(part 1 of 2)
# Autodesk Inventor assembly: Raspberry Pi 3
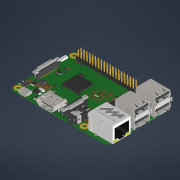
[picture p0: Inventor's stored thumbnail of the model, 180x180]
Saved by Autodesk Inventor 2021 (Build 250183000, 183)
## iProperties
Created: 2016-07-31
Part Number: Raspberry Pi 3
Document SubType Name: Assembly
Designer: sbahn
Author: sbahn
Sending System: SolidWorks 2016
Last Author: awillame
Last Saved: 2017-12-17
## Documents named in this file (329)
- C:\Users\sbahn\Desktop\개인자료\Workspace\Python Workspace\고등학교 졸업과제\2학기\modeling\electronic_file\raspi\Raspberry Pi 3.iam
- C:\Users\sbahn\Desktop\개인자료\Workspace\Python Workspace\고등학교 졸업과제\2학기\modeling\electronic_file\raspi\Raspberry Pi 3157.ipt
- C:\Users\sbahn\Desktop\개인자료\Workspace\Python Workspace\고등학교 졸업과제\2학기\modeling\electronic_file\raspi\Raspberry Pi 3242.ipt
- C:\Users\sbahn\Desktop\개인자료\Workspace\Python Workspace\고등학교 졸업과제\2학기\modeling\electronic_file\raspi\Raspberry Pi 3266.ipt
- C:\Users\sbahn\Desktop\개인자료\Workspace\Python Workspace\고등학교 졸업과제\2학기\modeling\electronic_file\raspi\raspberry_pi_3(bar_180_2x20).ipt
- C:\Users\sbahn\Desktop\개인자료\Workspace\Python Workspace\고등학교 졸업과제\2학기\modeling\electronic_file\raspi\RPi3_ModelB v1.iam
- C:\Users\sbahn\Desktop\개인자료\Workspace\Python Workspace\고등학교 졸업과제\2학기\modeling\electronic_file\raspi\Raspberry Pi 312.ipt
- C:\Users\sbahn\Desktop\개인자료\Workspace\Python Workspace\고등학교 졸업과제\2학기\modeling\electronic_file\raspi\Raspberry Pi 314.ipt
- C:\Users\sbahn\Desktop\개인자료\Workspace\Python Workspace\고등학교 졸업과제\2학기\modeling\electronic_file\raspi\Raspberry Pi 3172.ipt
- C:\Users\sbahn\Desktop\개인자료\Workspace\Python Workspace\고등학교 졸업과제\2학기\modeling\electronic_file\raspi\Raspberry Pi 3173.ipt
- C:\Users\sbahn\Desktop\개인자료\Workspace\Python Workspace\고등학교 졸업과제\2학기\modeling\electronic_file\raspi\Raspberry Pi 3174.ipt
- C:\Users\sbahn\Desktop\개인자료\Workspace\Python Workspace\고등학교 졸업과제\2학기\modeling\electronic_file\raspi\Raspberry Pi 3175.ipt
- C:\Users\sbahn\Desktop\개인자료\Workspace\Python Workspace\고등학교 졸업과제\2학기\modeling\electronic_file\raspi\Raspberry Pi 3176.ipt
- C:\Users\sbahn\Desktop\개인자료\Workspace\Python Workspace\고등학교 졸업과제\2학기\modeling\electronic_file\raspi\Raspberry Pi 3177.ipt
- C:\Users\sbahn\Desktop\개인자료\Workspace\Python Workspace\고등학교 졸업과제\2학기\modeling\electronic_file\raspi\Raspberry Pi 3178.ipt
- C:\Users\sbahn\Desktop\개인자료\Workspace\Python Workspace\고등학교 졸업과제\2학기\modeling\electronic_file\raspi\Raspberry Pi 3179.ipt
- C:\Users\sbahn\Desktop\개인자료\Workspace\Python Workspace\고등학교 졸업과제\2학기\modeling\electronic_file\raspi\Raspberry Pi 3180.ipt
- C:\Users\sbahn\Desktop\개인자료\Workspace\Python Workspace\고등학교 졸업과제\2학기\modeling\electronic_file\raspi\Raspberry Pi 3181.ipt
- C:\Users\sbahn\Desktop\개인자료\Workspace\Python Workspace\고등학교 졸업과제\2학기\modeling\electronic_file\raspi\Raspberry Pi 3182.ipt
- C:\Users\sbahn\Desktop\개인자료\Workspace\Python Workspace\고등학교 졸업과제\2학기\modeling\electronic_file\raspi\Raspberry Pi 3183.ipt
- C:\Users\sbahn\Desktop\개인자료\Workspace\Python Workspace\고등학교 졸업과제\2학기\modeling\electronic_file\raspi\Raspberry Pi 3184.ipt
- C:\Users\sbahn\Desktop\개인자료\Workspace\Python Workspace\고등학교 졸업과제\2학기\modeling\electronic_file\raspi\Raspberry Pi 3185.ipt
- C:\Users\sbahn\Desktop\개인자료\Workspace\Python Workspace\고등학교 졸업과제\2학기\modeling\electronic_file\raspi\Raspberry Pi 3186.ipt
- C:\Users\sbahn\Desktop\개인자료\Workspace\Python Workspace\고등학교 졸업과제\2학기\modeling\electronic_file\raspi\Raspberry Pi 3187.ipt
- C:\Users\sbahn\Desktop\개인자료\Workspace\Python Workspace\고등학교 졸업과제\2학기\modeling\electronic_file\raspi\Raspberry Pi 3188.ipt
- C:\Users\sbahn\Desktop\개인자료\Workspace\Python Workspace\고등학교 졸업과제\2학기\modeling\electronic_file\raspi\Raspberry Pi 3189.ipt
- C:\Users\sbahn\Desktop\개인자료\Workspace\Python Workspace\고등학교 졸업과제\2학기\modeling\electronic_file\raspi\Raspberry Pi 3190.ipt
- C:\Users\sbahn\Desktop\개인자료\Workspace\Python Workspace\고등학교 졸업과제\2학기\modeling\electronic_file\raspi\Raspberry Pi 3191.ipt
- C:\Users\sbahn\Desktop\개인자료\Workspace\Python Workspace\고등학교 졸업과제\2학기\modeling\electronic_file\raspi\Raspberry Pi 3192.ipt
- C:\Users\sbahn\Desktop\개인자료\Workspace\Python Workspace\고등학교 졸업과제\2학기\modeling\electronic_file\raspi\Raspberry Pi 3193.ipt
- C:\Users\sbahn\Desktop\개인자료\Workspace\Python Workspace\고등학교 졸업과제\2학기\modeling\electronic_file\raspi\Raspberry Pi 3194.ipt
- C:\Users\sbahn\Desktop\개인자료\Workspace\Python Workspace\고등학교 졸업과제\2학기\modeling\electronic_file\raspi\Raspberry Pi 3195.ipt
- C:\Users\sbahn\Desktop\개인자료\Workspace\Python Workspace\고등학교 졸업과제\2학기\modeling\electronic_file\raspi\Raspberry Pi 3196.ipt
- C:\Users\sbahn\Desktop\개인자료\Workspace\Python Workspace\고등학교 졸업과제\2학기\modeling\electronic_file\raspi\Raspberry Pi 3197.ipt
- C:\Users\sbahn\Desktop\개인자료\Workspace\Python Workspace\고등학교 졸업과제\2학기\modeling\electronic_file\raspi\Raspberry Pi 3198.ipt
- C:\Users\sbahn\Desktop\개인자료\Workspace\Python Workspace\고등학교 졸업과제\2학기\modeling\electronic_file\raspi\Raspberry Pi 3199.ipt
- C:\Users\sbahn\Desktop\개인자료\Workspace\Python Workspace\고등학교 졸업과제\2학기\modeling\electronic_file\raspi\Raspberry Pi 3200.ipt
- C:\Users\sbahn\Desktop\개인자료\Workspace\Python Workspace\고등학교 졸업과제\2학기\modeling\electronic_file\raspi\Raspberry Pi 3201.ipt
- C:\Users\sbahn\Desktop\개인자료\Workspace\Python Workspace\고등학교 졸업과제\2학기\modeling\electronic_file\raspi\Raspberry Pi 3202.ipt
- C:\Users\sbahn\Desktop\개인자료\Workspace\Python Workspace\고등학교 졸업과제\2학기\modeling\electronic_file\raspi\Raspberry Pi 3203.ipt
- C:\Users\sbahn\Desktop\개인자료\Workspace\Python Workspace\고등학교 졸업과제\2학기\modeling\electronic_file\raspi\Raspberry Pi 3204.ipt
- C:\Users\sbahn\Desktop\개인자료\Workspace\Python Workspace\고등학교 졸업과제\2학기\modeling\electronic_file\raspi\Raspberry Pi 3205.ipt
- C:\Users\sbahn\Desktop\개인자료\Workspace\Python Workspace\고등학교 졸업과제\2학기\modeling\electronic_file\raspi\Raspberry Pi 3206.ipt
- C:\Users\sbahn\Desktop\개인자료\Workspace\Python Workspace\고등학교 졸업과제\2학기\modeling\electronic_file\raspi\Raspberry Pi 3207.ipt
- C:\Users\sbahn\Desktop\개인자료\Workspace\Python Workspace\고등학교 졸업과제\2학기\modeling\electronic_file\raspi\Raspberry Pi 3208.ipt
- C:\Users\sbahn\Desktop\개인자료\Workspace\Python Workspace\고등학교 졸업과제\2학기\modeling\electronic_file\raspi\Raspberry Pi 3209.ipt
- C:\Users\sbahn\Desktop\개인자료\Workspace\Python Workspace\고등학교 졸업과제\2학기\modeling\electronic_file\raspi\Raspberry Pi 3210.ipt
- C:\Users\sbahn\Desktop\개인자료\Workspace\Python Workspace\고등학교 졸업과제\2학기\modeling\electronic_file\raspi\Raspberry Pi 3211.ipt
- C:\Users\sbahn\Desktop\개인자료\Workspace\Python Workspace\고등학교 졸업과제\2학기\modeling\electronic_file\raspi\Raspberry Pi 3212.ipt
- C:\Users\sbahn\Desktop\개인자료\Workspace\Python Workspace\고등학교 졸업과제\2학기\modeling\electronic_file\raspi\Raspberry Pi 3213.ipt
- C:\Users\sbahn\Desktop\개인자료\Workspace\Python Workspace\고등학교 졸업과제\2학기\modeling\electronic_file\raspi\Raspberry Pi 3214.ipt
- C:\Users\sbahn\Desktop\개인자료\Workspace\Python Workspace\고등학교 졸업과제\2학기\modeling\electronic_file\raspi\Raspberry Pi 3215.ipt
- C:\Users\sbahn\Desktop\개인자료\Workspace\Python Workspace\고등학교 졸업과제\2학기\modeling\electronic_file\raspi\Raspberry Pi 3216.ipt
- C:\Users\sbahn\Desktop\개인자료\Workspace\Python Workspace\고등학교 졸업과제\2학기\modeling\electronic_file\raspi\Raspberry Pi 3217.ipt
- C:\Users\sbahn\Desktop\개인자료\Workspace\Python Workspace\고등학교 졸업과제\2학기\modeling\electronic_file\raspi\Raspberry Pi 3218.ipt
- C:\Users\sbahn\Desktop\개인자료\Workspace\Python Workspace\고등학교 졸업과제\2학기\modeling\electronic_file\raspi\Raspberry Pi 3219.ipt
- C:\Users\sbahn\Desktop\개인자료\Workspace\Python Workspace\고등학교 졸업과제\2학기\modeling\electronic_file\raspi\Raspberry Pi 3220.ipt
- C:\Users\sbahn\Desktop\개인자료\Workspace\Python Workspace\고등학교 졸업과제\2학기\modeling\electronic_file\raspi\Raspberry Pi 3221.ipt
- C:\Users\sbahn\Desktop\개인자료\Workspace\Python Workspace\고등학교 졸업과제\2학기\modeling\electronic_file\raspi\Raspberry Pi 3222.ipt
- C:\Users\sbahn\Desktop\개인자료\Workspace\Python Workspace\고등학교 졸업과제\2학기\modeling\electronic_file\raspi\Raspberry Pi 3223.ipt
- C:\Users\sbahn\Desktop\개인자료\Workspace\Python Workspace\고등학교 졸업과제\2학기\modeling\electronic_file\raspi\Raspberry Pi 3224.ipt
- C:\Users\sbahn\Desktop\개인자료\Workspace\Python Workspace\고등학교 졸업과제\2학기\modeling\electronic_file\raspi\Raspberry Pi 3225.ipt
- C:\Users\sbahn\Desktop\개인자료\Workspace\Python Workspace\고등학교 졸업과제\2학기\modeling\electronic_file\raspi\Raspberry Pi 3226.ipt
- C:\Users\sbahn\Desktop\개인자료\Workspace\Python Workspace\고등학교 졸업과제\2학기\modeling\electronic_file\raspi\Raspberry Pi 3227.ipt
- C:\Users\sbahn\Desktop\개인자료\Workspace\Python Workspace\고등학교 졸업과제\2학기\modeling\electronic_file\raspi\Raspberry Pi 3228.ipt
- C:\Users\sbahn\Desktop\개인자료\Workspace\Python Workspace\고등학교 졸업과제\2학기\modeling\electronic_file\raspi\Raspberry Pi 3229.ipt
- C:\Users\sbahn\Desktop\개인자료\Workspace\Python Workspace\고등학교 졸업과제\2학기\modeling\electronic_file\raspi\Raspberry Pi 3230.ipt
- C:\Users\sbahn\Desktop\개인자료\Workspace\Python Workspace\고등학교 졸업과제\2학기\modeling\electronic_file\raspi\Raspberry Pi 3231.ipt
- C:\Users\sbahn\Desktop\개인자료\Workspace\Python Workspace\고등학교 졸업과제\2학기\modeling\electronic_file\raspi\Raspberry Pi 3232.ipt
- C:\Users\sbahn\Desktop\개인자료\Workspace\Python Workspace\고등학교 졸업과제\2학기\modeling\electronic_file\raspi\Raspberry Pi 3233.ipt
- C:\Users\sbahn\Desktop\개인자료\Workspace\Python Workspace\고등학교 졸업과제\2학기\modeling\electronic_file\raspi\Raspberry Pi 3234.ipt
- C:\Users\sbahn\Desktop\개인자료\Workspace\Python Workspace\고등학교 졸업과제\2학기\modeling\electronic_file\raspi\Raspberry Pi 3235.ipt
- C:\Users\sbahn\Desktop\개인자료\Workspace\Python Workspace\고등학교 졸업과제\2학기\modeling\electronic_file\raspi\Raspberry Pi 31.ipt
- C:\Users\sbahn\Desktop\개인자료\Workspace\Python Workspace\고등학교 졸업과제\2학기\modeling\electronic_file\raspi\Raspberry Pi 36.ipt
- C:\Users\sbahn\Desktop\개인자료\Workspace\Python Workspace\고등학교 졸업과제\2학기\modeling\electronic_file\raspi\Raspberry Pi 32.ipt
- C:\Users\sbahn\Desktop\개인자료\Workspace\Python Workspace\고등학교 졸업과제\2학기\modeling\electronic_file\raspi\Raspberry Pi 33.ipt
- C:\Users\sbahn\Desktop\개인자료\Workspace\Python Workspace\고등학교 졸업과제\2학기\modeling\electronic_file\raspi\Raspberry Pi 34.ipt
- C:\Users\sbahn\Desktop\개인자료\Workspace\Python Workspace\고등학교 졸업과제\2학기\modeling\electronic_file\raspi\Raspberry Pi 35.ipt
- C:\Users\sbahn\Desktop\개인자료\Workspace\Python Workspace\고등학교 졸업과제\2학기\modeling\electronic_file\raspi\Raspberry Pi 37.ipt
- C:\Users\sbahn\Desktop\개인자료\Workspace\Python Workspace\고등학교 졸업과제\2학기\modeling\electronic_file\raspi\Raspberry Pi 38.ipt
- C:\Users\sbahn\Desktop\개인자료\Workspace\Python Workspace\고등학교 졸업과제\2학기\modeling\electronic_file\raspi\Raspberry Pi 39.ipt
- C:\Users\sbahn\Desktop\개인자료\Workspace\Python Workspace\고등학교 졸업과제\2학기\modeling\electronic_file\raspi\Raspberry Pi 310.ipt
- C:\Users\sbahn\Desktop\개인자료\Workspace\Python Workspace\고등학교 졸업과제\2학기\modeling\electronic_file\raspi\Raspberry Pi 311.ipt
- C:\Users\sbahn\Desktop\개인자료\Workspace\Python Workspace\고등학교 졸업과제\2학기\modeling\electronic_file\raspi\Raspberry Pi 313.ipt
- C:\Users\sbahn\Desktop\개인자료\Workspace\Python Workspace\고등학교 졸업과제\2학기\modeling\electronic_file\raspi\Raspberry Pi 315.ipt
- C:\Users\sbahn\Desktop\개인자료\Workspace\Python Workspace\고등학교 졸업과제\2학기\modeling\electronic_file\raspi\Raspberry Pi 316.ipt
- C:\Users\sbahn\Desktop\개인자료\Workspace\Python Workspace\고등학교 졸업과제\2학기\modeling\electronic_file\raspi\Raspberry Pi 317.ipt
- C:\Users\sbahn\Desktop\개인자료\Workspace\Python Workspace\고등학교 졸업과제\2학기\modeling\electronic_file\raspi\Raspberry Pi 318.ipt
- C:\Users\sbahn\Desktop\개인자료\Workspace\Python Workspace\고등학교 졸업과제\2학기\modeling\electronic_file\raspi\Raspberry Pi 319.ipt
- C:\Users\sbahn\Desktop\개인자료\Workspace\Python Workspace\고등학교 졸업과제\2학기\modeling\electronic_file\raspi\Raspberry Pi 320.ipt
- C:\Users\sbahn\Desktop\개인자료\Workspace\Python Workspace\고등학교 졸업과제\2학기\modeling\electronic_file\raspi\Raspberry Pi 322.ipt
- C:\Users\sbahn\Desktop\개인자료\Workspace\Python Workspace\고등학교 졸업과제\2학기\modeling\electronic_file\raspi\Raspberry Pi 323.ipt
- C:\Users\sbahn\Desktop\개인자료\Workspace\Python Workspace\고등학교 졸업과제\2학기\modeling\electronic_file\raspi\Raspberry Pi 324.ipt
- C:\Users\sbahn\Desktop\개인자료\Workspace\Python Workspace\고등학교 졸업과제\2학기\modeling\electronic_file\raspi\Raspberry Pi 325.ipt
- C:\Users\sbahn\Desktop\개인자료\Workspace\Python Workspace\고등학교 졸업과제\2학기\modeling\electronic_file\raspi\Raspberry Pi 326.ipt
- C:\Users\sbahn\Desktop\개인자료\Workspace\Python Workspace\고등학교 졸업과제\2학기\modeling\electronic_file\raspi\Raspberry Pi 327.ipt
- C:\Users\sbahn\Desktop\개인자료\Workspace\Python Workspace\고등학교 졸업과제\2학기\modeling\electronic_file\raspi\Raspberry Pi 328.ipt
- C:\Users\sbahn\Desktop\개인자료\Workspace\Python Workspace\고등학교 졸업과제\2학기\modeling\electronic_file\raspi\Raspberry Pi 329.ipt
- C:\Users\sbahn\Desktop\개인자료\Workspace\Python Workspace\고등학교 졸업과제\2학기\modeling\electronic_file\raspi\Raspberry Pi 330.ipt
- C:\Users\sbahn\Desktop\개인자료\Workspace\Python Workspace\고등학교 졸업과제\2학기\modeling\electronic_file\raspi\Raspberry Pi 331.ipt
- C:\Users\sbahn\Desktop\개인자료\Workspace\Python Workspace\고등학교 졸업과제\2학기\modeling\electronic_file\raspi\Raspberry Pi 332.ipt
- C:\Users\sbahn\Desktop\개인자료\Workspace\Python Workspace\고등학교 졸업과제\2학기\modeling\electronic_file\raspi\Raspberry Pi 333.ipt
- C:\Users\sbahn\Desktop\개인자료\Workspace\Python Workspace\고등학교 졸업과제\2학기\modeling\electronic_file\raspi\Raspberry Pi 334.ipt
- C:\Users\sbahn\Desktop\개인자료\Workspace\Python Workspace\고등학교 졸업과제\2학기\modeling\electronic_file\raspi\Raspberry Pi 335.ipt
- C:\Users\sbahn\Desktop\개인자료\Workspace\Python Workspace\고등학교 졸업과제\2학기\modeling\electronic_file\raspi\Raspberry Pi 336.ipt
- C:\Users\sbahn\Desktop\개인자료\Workspace\Python Workspace\고등학교 졸업과제\2학기\modeling\electronic_file\raspi\Raspberry Pi 337.ipt
- C:\Users\sbahn\Desktop\개인자료\Workspace\Python Workspace\고등학교 졸업과제\2학기\modeling\electronic_file\raspi\Raspberry Pi 338.ipt
- C:\Users\sbahn\Desktop\개인자료\Workspace\Python Workspace\고등학교 졸업과제\2학기\modeling\electronic_file\raspi\Raspberry Pi 339.ipt
- C:\Users\sbahn\Desktop\개인자료\Workspace\Python Workspace\고등학교 졸업과제\2학기\modeling\electronic_file\raspi\Raspberry Pi 340.ipt
- C:\Users\sbahn\Desktop\개인자료\Workspace\Python Workspace\고등학교 졸업과제\2학기\modeling\electronic_file\raspi\Raspberry Pi 341.ipt
- C:\Users\sbahn\Desktop\개인자료\Workspace\Python Workspace\고등학교 졸업과제\2학기\modeling\electronic_file\raspi\Raspberry Pi 342.ipt
- C:\Users\sbahn\Desktop\개인자료\Workspace\Python Workspace\고등학교 졸업과제\2학기\modeling\electronic_file\raspi\Raspberry Pi 343.ipt
- C:\Users\sbahn\Desktop\개인자료\Workspace\Python Workspace\고등학교 졸업과제\2학기\modeling\electronic_file\raspi\Raspberry Pi 344.ipt
- C:\Users\sbahn\Desktop\개인자료\Workspace\Python Workspace\고등학교 졸업과제\2학기\modeling\electronic_file\raspi\Raspberry Pi 345.ipt
- C:\Users\sbahn\Desktop\개인자료\Workspace\Python Workspace\고등학교 졸업과제\2학기\modeling\electronic_file\raspi\Raspberry Pi 346.ipt
- C:\Users\sbahn\Desktop\개인자료\Workspace\Python Workspace\고등학교 졸업과제\2학기\modeling\electronic_file\raspi\Raspberry Pi 347.ipt
- C:\Users\sbahn\Desktop\개인자료\Workspace\Python Workspace\고등학교 졸업과제\2학기\modeling\electronic_file\raspi\Raspberry Pi 348.ipt
- C:\Users\sbahn\Desktop\개인자료\Workspace\Python Workspace\고등학교 졸업과제\2학기\modeling\electronic_file\raspi\Raspberry Pi 349.ipt
- C:\Users\sbahn\Desktop\개인자료\Workspace\Python Workspace\고등학교 졸업과제\2학기\modeling\electronic_file\raspi\Raspberry Pi 350.ipt
- C:\Users\sbahn\Desktop\개인자료\Workspace\Python Workspace\고등학교 졸업과제\2학기\modeling\electronic_file\raspi\Raspberry Pi 351.ipt
- C:\Users\sbahn\Desktop\개인자료\Workspace\Python Workspace\고등학교 졸업과제\2학기\modeling\electronic_file\raspi\Raspberry Pi 352.ipt
- C:\Users\sbahn\Desktop\개인자료\Workspace\Python Workspace\고등학교 졸업과제\2학기\modeling\electronic_file\raspi\Raspberry Pi 353.ipt
- C:\Users\sbahn\Desktop\개인자료\Workspace\Python Workspace\고등학교 졸업과제\2학기\modeling\electronic_file\raspi\Raspberry Pi 354.ipt
- C:\Users\sbahn\Desktop\개인자료\Workspace\Python Workspace\고등학교 졸업과제\2학기\modeling\electronic_file\raspi\Raspberry Pi 355.ipt
- C:\Users\sbahn\Desktop\개인자료\Workspace\Python Workspace\고등학교 졸업과제\2학기\modeling\electronic_file\raspi\Raspberry Pi 356.ipt
- C:\Users\sbahn\Desktop\개인자료\Workspace\Python Workspace\고등학교 졸업과제\2학기\modeling\electronic_file\raspi\Raspberry Pi 357.ipt
- C:\Users\sbahn\Desktop\개인자료\Workspace\Python Workspace\고등학교 졸업과제\2학기\modeling\electronic_file\raspi\Raspberry Pi 358.ipt
- C:\Users\sbahn\Desktop\개인자료\Workspace\Python Workspace\고등학교 졸업과제\2학기\modeling\electronic_file\raspi\Raspberry Pi 359.ipt
- C:\Users\sbahn\Desktop\개인자료\Workspace\Python Workspace\고등학교 졸업과제\2학기\modeling\electronic_file\raspi\Raspberry Pi 360.ipt
- C:\Users\sbahn\Desktop\개인자료\Workspace\Python Workspace\고등학교 졸업과제\2학기\modeling\electronic_file\raspi\Raspberry Pi 361.ipt
- C:\Users\sbahn\Desktop\개인자료\Workspace\Python Workspace\고등학교 졸업과제\2학기\modeling\electronic_file\raspi\Raspberry Pi 362.ipt
- C:\Users\sbahn\Desktop\개인자료\Workspace\Python Workspace\고등학교 졸업과제\2학기\modeling\electronic_file\raspi\Raspberry Pi 363.ipt
- C:\Users\sbahn\Desktop\개인자료\Workspace\Python Workspace\고등학교 졸업과제\2학기\modeling\electronic_file\raspi\Raspberry Pi 364.ipt
- C:\Users\sbahn\Desktop\개인자료\Workspace\Python Workspace\고등학교 졸업과제\2학기\modeling\electronic_file\raspi\Raspberry Pi 365.ipt
- C:\Users\sbahn\Desktop\개인자료\Workspace\Python Workspace\고등학교 졸업과제\2학기\modeling\electronic_file\raspi\Raspberry Pi 366.ipt
- C:\Users\sbahn\Desktop\개인자료\Workspace\Python Workspace\고등학교 졸업과제\2학기\modeling\electronic_file\raspi\Raspberry Pi 367.ipt
- C:\Users\sbahn\Desktop\개인자료\Workspace\Python Workspace\고등학교 졸업과제\2학기\modeling\electronic_file\raspi\Raspberry Pi 368.ipt
- C:\Users\sbahn\Desktop\개인자료\Workspace\Python Workspace\고등학교 졸업과제\2학기\modeling\electronic_file\raspi\Raspberry Pi 369.ipt
- C:\Users\sbahn\Desktop\개인자료\Workspace\Python Workspace\고등학교 졸업과제\2학기\modeling\electronic_file\raspi\Raspberry Pi 370.ipt
- C:\Users\sbahn\Desktop\개인자료\Workspace\Python Workspace\고등학교 졸업과제\2학기\modeling\electronic_file\raspi\Raspberry Pi 371.ipt
- C:\Users\sbahn\Desktop\개인자료\Workspace\Python Workspace\고등학교 졸업과제\2학기\modeling\electronic_file\raspi\Raspberry Pi 372.ipt
- C:\Users\sbahn\Desktop\개인자료\Workspace\Python Workspace\고등학교 졸업과제\2학기\modeling\electronic_file\raspi\Raspberry Pi 373.ipt
- C:\Users\sbahn\Desktop\개인자료\Workspace\Python Workspace\고등학교 졸업과제\2학기\modeling\electronic_file\raspi\Raspberry Pi 374.ipt
- C:\Users\sbahn\Desktop\개인자료\Workspace\Python Workspace\고등학교 졸업과제\2학기\modeling\electronic_file\raspi\Raspberry Pi 375.ipt
- C:\Users\sbahn\Desktop\개인자료\Workspace\Python Workspace\고등학교 졸업과제\2학기\modeling\electronic_file\raspi\Raspberry Pi 376.ipt
- C:\Users\sbahn\Desktop\개인자료\Workspace\Python Workspace\고등학교 졸업과제\2학기\modeling\electronic_file\raspi\Raspberry Pi 377.ipt
- C:\Users\sbahn\Desktop\개인자료\Workspace\Python Workspace\고등학교 졸업과제\2학기\modeling\electronic_file\raspi\Raspberry Pi 378.ipt
- C:\Users\sbahn\Desktop\개인자료\Workspace\Python Workspace\고등학교 졸업과제\2학기\modeling\electronic_file\raspi\Raspberry Pi 379.ipt
- C:\Users\sbahn\Desktop\개인자료\Workspace\Python Workspace\고등학교 졸업과제\2학기\modeling\electronic_file\raspi\Raspberry Pi 380.ipt
- C:\Users\sbahn\Desktop\개인자료\Workspace\Python Workspace\고등학교 졸업과제\2학기\modeling\electronic_file\raspi\Raspberry Pi 381.ipt
- C:\Users\sbahn\Desktop\개인자료\Workspace\Python Workspace\고등학교 졸업과제\2학기\modeling\electronic_file\raspi\Raspberry Pi 382.ipt
- C:\Users\sbahn\Desktop\개인자료\Workspace\Python Workspace\고등학교 졸업과제\2학기\modeling\electronic_file\raspi\Raspberry Pi 383.ipt
- C:\Users\sbahn\Desktop\개인자료\Workspace\Python Workspace\고등학교 졸업과제\2학기\modeling\electronic_file\raspi\Raspberry Pi 385.ipt
- C:\Users\sbahn\Desktop\개인자료\Workspace\Python Workspace\고등학교 졸업과제\2학기\modeling\electronic_file\raspi\Raspberry Pi 386.ipt
- C:\Users\sbahn\Desktop\개인자료\Workspace\Python Workspace\고등학교 졸업과제\2학기\modeling\electronic_file\raspi\Raspberry Pi 387.ipt
- C:\Users\sbahn\Desktop\개인자료\Workspace\Python Workspace\고등학교 졸업과제\2학기\modeling\electronic_file\raspi\Raspberry Pi 388.ipt
- C:\Users\sbahn\Desktop\개인자료\Workspace\Python Workspace\고등학교 졸업과제\2학기\modeling\electronic_file\raspi\Raspberry Pi 390.ipt
- C:\Users\sbahn\Desktop\개인자료\Workspace\Python Workspace\고등학교 졸업과제\2학기\modeling\electronic_file\raspi\Raspberry Pi 391.ipt
- C:\Users\sbahn\Desktop\개인자료\Workspace\Python Workspace\고등학교 졸업과제\2학기\modeling\electronic_file\raspi\Raspberry Pi 393.ipt
- C:\Users\sbahn\Desktop\개인자료\Workspace\Python Workspace\고등학교 졸업과제\2학기\modeling\electronic_file\raspi\Raspberry Pi 394.ipt
- C:\Users\sbahn\Desktop\개인자료\Workspace\Python Workspace\고등학교 졸업과제\2학기\modeling\electronic_file\raspi\Raspberry Pi 395.ipt
- C:\Users\sbahn\Desktop\개인자료\Workspace\Python Workspace\고등학교 졸업과제\2학기\modeling\electronic_file\raspi\Raspberry Pi 396.ipt
- C:\Users\sbahn\Desktop\개인자료\Workspace\Python Workspace\고등학교 졸업과제\2학기\modeling\electronic_file\raspi\Raspberry Pi 397.ipt
- C:\Users\sbahn\Desktop\개인자료\Workspace\Python Workspace\고등학교 졸업과제\2학기\modeling\electronic_file\raspi\Raspberry Pi 398.ipt
- C:\Users\sbahn\Desktop\개인자료\Workspace\Python Workspace\고등학교 졸업과제\2학기\modeling\electronic_file\raspi\Raspberry Pi 399.ipt
- C:\Users\sbahn\Desktop\개인자료\Workspace\Python Workspace\고등학교 졸업과제\2학기\modeling\electronic_file\raspi\Raspberry Pi 3100.ipt
- C:\Users\sbahn\Desktop\개인자료\Workspace\Python Workspace\고등학교 졸업과제\2학기\modeling\electronic_file\raspi\Raspberry Pi 3101.ipt
- C:\Users\sbahn\Desktop\개인자료\Workspace\Python Workspace\고등학교 졸업과제\2학기\modeling\electronic_file\raspi\Raspberry Pi 3102.ipt
- C:\Users\sbahn\Desktop\개인자료\Workspace\Python Workspace\고등학교 졸업과제\2학기\modeling\electronic_file\raspi\Raspberry Pi 3103.ipt
- C:\Users\sbahn\Desktop\개인자료\Workspace\Python Workspace\고등학교 졸업과제\2학기\modeling\electronic_file\raspi\Raspberry Pi 3104.ipt
- C:\Users\sbahn\Desktop\개인자료\Workspace\Python Workspace\고등학교 졸업과제\2학기\modeling\electronic_file\raspi\Raspberry Pi 3105.ipt
- C:\Users\sbahn\Desktop\개인자료\Workspace\Python Workspace\고등학교 졸업과제\2학기\modeling\electronic_file\raspi\Raspberry Pi 3106.ipt
- C:\Users\sbahn\Desktop\개인자료\Workspace\Python Workspace\고등학교 졸업과제\2학기\modeling\electronic_file\raspi\Raspberry Pi 3107.ipt
- C:\Users\sbahn\Desktop\개인자료\Workspace\Python Workspace\고등학교 졸업과제\2학기\modeling\electronic_file\raspi\Raspberry Pi 3108.ipt
- C:\Users\sbahn\Desktop\개인자료\Workspace\Python Workspace\고등학교 졸업과제\2학기\modeling\electronic_file\raspi\Raspberry Pi 3109.ipt
- C:\Users\sbahn\Desktop\개인자료\Workspace\Python Workspace\고등학교 졸업과제\2학기\modeling\electronic_file\raspi\Raspberry Pi 3110.ipt
- C:\Users\sbahn\Desktop\개인자료\Workspace\Python Workspace\고등학교 졸업과제\2학기\modeling\electronic_file\raspi\Raspberry Pi 3111.ipt
- C:\Users\sbahn\Desktop\개인자료\Workspace\Python Workspace\고등학교 졸업과제\2학기\modeling\electronic_file\raspi\Raspberry Pi 3112.ipt
- C:\Users\sbahn\Desktop\개인자료\Workspace\Python Workspace\고등학교 졸업과제\2학기\modeling\electronic_file\raspi\Raspberry Pi 3113.ipt
- C:\Users\sbahn\Desktop\개인자료\Workspace\Python Workspace\고등학교 졸업과제\2학기\modeling\electronic_file\raspi\Raspberry Pi 3114.ipt
- C:\Users\sbahn\Desktop\개인자료\Workspace\Python Workspace\고등학교 졸업과제\2학기\modeling\electronic_file\raspi\Raspberry Pi 3115.ipt
- C:\Users\sbahn\Desktop\개인자료\Workspace\Python Workspace\고등학교 졸업과제\2학기\modeling\electronic_file\raspi\Raspberry Pi 3116.ipt
- C:\Users\sbahn\Desktop\개인자료\Workspace\Python Workspace\고등학교 졸업과제\2학기\modeling\electronic_file\raspi\Raspberry Pi 3117.ipt
- C:\Users\sbahn\Desktop\개인자료\Workspace\Python Workspace\고등학교 졸업과제\2학기\modeling\electronic_file\raspi\Raspberry Pi 3118.ipt
- C:\Users\sbahn\Desktop\개인자료\Workspace\Python Workspace\고등학교 졸업과제\2학기\modeling\electronic_file\raspi\Raspberry Pi 3119.ipt
- C:\Users\sbahn\Desktop\개인자료\Workspace\Python Workspace\고등학교 졸업과제\2학기\modeling\electronic_file\raspi\Raspberry Pi 3120.ipt
- C:\Users\sbahn\Desktop\개인자료\Workspace\Python Workspace\고등학교 졸업과제\2학기\modeling\electronic_file\raspi\Raspberry Pi 3121.ipt
- C:\Users\sbahn\Desktop\개인자료\Workspace\Python Workspace\고등학교 졸업과제\2학기\modeling\electronic_file\raspi\Raspberry Pi 3122.ipt
- C:\Users\sbahn\Desktop\개인자료\Workspace\Python Workspace\고등학교 졸업과제\2학기\modeling\electronic_file\raspi\Raspberry Pi 3123.ipt
- C:\Users\sbahn\Desktop\개인자료\Workspace\Python Workspace\고등학교 졸업과제\2학기\modeling\electronic_file\raspi\Raspberry Pi 3124.ipt
- C:\Users\sbahn\Desktop\개인자료\Workspace\Python Workspace\고등학교 졸업과제\2학기\modeling\electronic_file\raspi\Raspberry Pi 3125.ipt
- C:\Users\sbahn\Desktop\개인자료\Workspace\Python Workspace\고등학교 졸업과제\2학기\modeling\electronic_file\raspi\Raspberry Pi 3126.ipt
- C:\Users\sbahn\Desktop\개인자료\Workspace\Python Workspace\고등학교 졸업과제\2학기\modeling\electronic_file\raspi\Raspberry Pi 3127.ipt
- C:\Users\sbahn\Desktop\개인자료\Workspace\Python Workspace\고등학교 졸업과제\2학기\modeling\electronic_file\raspi\Raspberry Pi 3128.ipt
- C:\Users\sbahn\Desktop\개인자료\Workspace\Python Workspace\고등학교 졸업과제\2학기\modeling\electronic_file\raspi\Raspberry Pi 3129.ipt
- C:\Users\sbahn\Desktop\개인자료\Workspace\Python Workspace\고등학교 졸업과제\2학기\modeling\electronic_file\raspi\Raspberry Pi 3130.ipt
- C:\Users\sbahn\Desktop\개인자료\Workspace\Python Workspace\고등학교 졸업과제\2학기\modeling\electronic_file\raspi\Raspberry Pi 3131.ipt
- C:\Users\sbahn\Desktop\개인자료\Workspace\Python Workspace\고등학교 졸업과제\2학기\modeling\electronic_file\raspi\Raspberry Pi 3132.ipt
- C:\Users\sbahn\Desktop\개인자료\Workspace\Python Workspace\고등학교 졸업과제\2학기\modeling\electronic_file\raspi\Raspberry Pi 3133.ipt
- C:\Users\sbahn\Desktop\개인자료\Workspace\Python Workspace\고등학교 졸업과제\2학기\modeling\electronic_file\raspi\Raspberry Pi 3134.ipt
- C:\Users\sbahn\Desktop\개인자료\Workspace\Python Workspace\고등학교 졸업과제\2학기\modeling\electronic_file\raspi\Raspberry Pi 3135.ipt
- C:\Users\sbahn\Desktop\개인자료\Workspace\Python Workspace\고등학교 졸업과제\2학기\modeling\electronic_file\raspi\Raspberry Pi 3137.ipt
- C:\Users\sbahn\Desktop\개인자료\Workspace\Python Workspace\고등학교 졸업과제\2학기\modeling\electronic_file\raspi\Raspberry Pi 3138.ipt
- C:\Users\sbahn\Desktop\개인자료\Workspace\Python Workspace\고등학교 졸업과제\2학기\modeling\electronic_file\raspi\Raspberry Pi 3139.ipt
- C:\Users\sbahn\Desktop\개인자료\Workspace\Python Workspace\고등학교 졸업과제\2학기\modeling\electronic_file\raspi\Raspberry Pi 3140.ipt
- C:\Users\sbahn\Desktop\개인자료\Workspace\Python Workspace\고등학교 졸업과제\2학기\modeling\electronic_file\raspi\Raspberry Pi 3141.ipt
- C:\Users\sbahn\Desktop\개인자료\Workspace\Python Workspace\고등학교 졸업과제\2학기\modeling\electronic_file\raspi\Raspberry Pi 3142.ipt
- C:\Users\sbahn\Desktop\개인자료\Workspace\Python Workspace\고등학교 졸업과제\2학기\modeling\electronic_file\raspi\Raspberry Pi 3143.ipt
- C:\Users\sbahn\Desktop\개인자료\Workspace\Python Workspace\고등학교 졸업과제\2학기\modeling\electronic_file\raspi\Raspberry Pi 3144.ipt
- C:\Users\sbahn\Desktop\개인자료\Workspace\Python Workspace\고등학교 졸업과제\2학기\modeling\electronic_file\raspi\Raspberry Pi 3146.ipt
- C:\Users\sbahn\Desktop\개인자료\Workspace\Python Workspace\고등학교 졸업과제\2학기\modeling\electronic_file\raspi\Raspberry Pi 3147.ipt
- C:\Users\sbahn\Desktop\개인자료\Workspace\Python Workspace\고등학교 졸업과제\2학기\modeling\electronic_file\raspi\Raspberry Pi 3149.ipt
- C:\Users\sbahn\Desktop\개인자료\Workspace\Python Workspace\고등학교 졸업과제\2학기\modeling\electronic_file\raspi\Raspberry Pi 3150.ipt
- C:\Users\sbahn\Desktop\개인자료\Workspace\Python Workspace\고등학교 졸업과제\2학기\modeling\electronic_file\raspi\Raspberry Pi 3151.ipt
- C:\Users\sbahn\Desktop\개인자료\Workspace\Python Workspace\고등학교 졸업과제\2학기\modeling\electronic_file\raspi\Raspberry Pi 3152.ipt
- C:\Users\sbahn\Desktop\개인자료\Workspace\Python Workspace\고등학교 졸업과제\2학기\modeling\electronic_file\raspi\Raspberry Pi 3153.ipt
- C:\Users\sbahn\Desktop\개인자료\Workspace\Python Workspace\고등학교 졸업과제\2학기\modeling\electronic_file\raspi\Raspberry Pi 3154.ipt
- C:\Users\sbahn\Desktop\개인자료\Workspace\Python Workspace\고등학교 졸업과제\2학기\modeling\electronic_file\raspi\Raspberry Pi 3155.ipt
- C:\Users\sbahn\Desktop\개인자료\Workspace\Python Workspace\고등학교 졸업과제\2학기\modeling\electronic_file\raspi\Raspberry Pi 3156.ipt
- C:\Users\sbahn\Desktop\개인자료\Workspace\Python Workspace\고등학교 졸업과제\2학기\modeling\electronic_file\raspi\Raspberry Pi 3158.ipt
- C:\Users\sbahn\Desktop\개인자료\Workspace\Python Workspace\고등학교 졸업과제\2학기\modeling\electronic_file\raspi\Raspberry Pi 3159.ipt
- C:\Users\sbahn\Desktop\개인자료\Workspace\Python Workspace\고등학교 졸업과제\2학기\modeling\electronic_file\raspi\Raspberry Pi 3160.ipt
- C:\Users\sbahn\Desktop\개인자료\Workspace\Python Workspace\고등학교 졸업과제\2학기\modeling\electronic_file\raspi\Raspberry Pi 3161.ipt
- C:\Users\sbahn\Desktop\개인자료\Workspace\Python Workspace\고등학교 졸업과제\2학기\modeling\electronic_file\raspi\Raspberry Pi 3162.ipt
- C:\Users\sbahn\Desktop\개인자료\Workspace\Python Workspace\고등학교 졸업과제\2학기\modeling\electronic_file\raspi\Raspberry Pi 3163.ipt
- C:\Users\sbahn\Desktop\개인자료\Workspace\Python Workspace\고등학교 졸업과제\2학기\modeling\electronic_file\raspi\Raspberry Pi 3164.ipt
- C:\Users\sbahn\Desktop\개인자료\Workspace\Python Workspace\고등학교 졸업과제\2학기\modeling\electronic_file\raspi\Raspberry Pi 3165.ipt
- C:\Users\sbahn\Desktop\개인자료\Workspace\Python Workspace\고등학교 졸업과제\2학기\modeling\electronic_file\raspi\Raspberry Pi 3166.ipt
- C:\Users\sbahn\Desktop\개인자료\Workspace\Python Workspace\고등학교 졸업과제\2학기\modeling\electronic_file\raspi\Raspberry Pi 3167.ipt
- C:\Users\sbahn\Desktop\개인자료\Workspace\Python Workspace\고등학교 졸업과제\2학기\modeling\electronic_file\raspi\Raspberry Pi 3168.ipt
- C:\Users\sbahn\Desktop\개인자료\Workspace\Python Workspace\고등학교 졸업과제\2학기\modeling\electronic_file\raspi\Raspberry Pi 3169.ipt
- C:\Users\sbahn\Desktop\개인자료\Workspace\Python Workspace\고등학교 졸업과제\2학기\modeling\electronic_file\raspi\Raspberry Pi 3170.ipt
- C:\Users\sbahn\Desktop\개인자료\Workspace\Python Workspace\고등학교 졸업과제\2학기\modeling\electronic_file\raspi\Raspberry Pi 3171.ipt
- C:\Users\sbahn\Desktop\개인자료\Workspace\Python Workspace\고등학교 졸업과제\2학기\modeling\electronic_file\raspi\Raspberry Pi 3276.ipt
- C:\Users\sbahn\Desktop\개인자료\Workspace\Python Workspace\고등학교 졸업과제\2학기\modeling\electronic_file\raspi\Raspberry Pi 3277.ipt
- C:\Users\sbahn\Desktop\개인자료\Workspace\Python Workspace\고등학교 졸업과제\2학기\modeling\electronic_file\raspi\Raspberry Pi 3278.ipt
- C:\Users\sbahn\Desktop\개인자료\Workspace\Python Workspace\고등학교 졸업과제\2학기\modeling\electronic_file\raspi\Raspberry Pi 3279.ipt
- C:\Users\sbahn\Desktop\개인자료\Workspace\Python Workspace\고등학교 졸업과제\2학기\modeling\electronic_file\raspi\Raspberry Pi 3280.ipt
- C:\Users\sbahn\Desktop\개인자료\Workspace\Python Workspace\고등학교 졸업과제\2학기\modeling\electronic_file\raspi\Raspberry Pi 3281.ipt
- C:\Users\sbahn\Desktop\개인자료\Workspace\Python Workspace\고등학교 졸업과제\2학기\modeling\electronic_file\raspi\Raspberry Pi 3282.ipt
- C:\Users\sbahn\Desktop\개인자료\Workspace\Python Workspace\고등학교 졸업과제\2학기\modeling\electronic_file\raspi\Raspberry Pi 3283.ipt
- C:\Users\sbahn\Desktop\개인자료\Workspace\Python Workspace\고등학교 졸업과제\2학기\modeling\electronic_file\raspi\Raspberry Pi 3284.ipt
- C:\Users\sbahn\Desktop\개인자료\Workspace\Python Workspace\고등학교 졸업과제\2학기\modeling\electronic_file\raspi\Raspberry Pi 3285.ipt
- C:\Users\sbahn\Desktop\개인자료\Workspace\Python Workspace\고등학교 졸업과제\2학기\modeling\electronic_file\raspi\Raspberry Pi 3286.ipt
- C:\Users\sbahn\Desktop\개인자료\Workspace\Python Workspace\고등학교 졸업과제\2학기\modeling\electronic_file\raspi\Raspberry Pi 3287.ipt
- C:\Users\sbahn\Desktop\개인자료\Workspace\Python Workspace\고등학교 졸업과제\2학기\modeling\electronic_file\raspi\Raspberry Pi 3288.ipt
- C:\Users\sbahn\Desktop\개인자료\Workspace\Python Workspace\고등학교 졸업과제\2학기\modeling\electronic_file\raspi\Raspberry Pi 3289.ipt
- C:\Users\sbahn\Desktop\개인자료\Workspace\Python Workspace\고등학교 졸업과제\2학기\modeling\electronic_file\raspi\Raspberry Pi 3290.ipt
- C:\Users\sbahn\Desktop\개인자료\Workspace\Python Workspace\고등학교 졸업과제\2학기\modeling\electronic_file\raspi\Raspberry Pi 3291.ipt
- C:\Users\sbahn\Desktop\개인자료\Workspace\Python Workspace\고등학교 졸업과제\2학기\modeling\electronic_file\raspi\Raspberry Pi 3292.ipt
- C:\Users\sbahn\Desktop\개인자료\Workspace\Python Workspace\고등학교 졸업과제\2학기\modeling\electronic_file\raspi\Raspberry Pi 3293.ipt
- C:\Users\sbahn\Desktop\개인자료\Workspace\Python Workspace\고등학교 졸업과제\2학기\modeling\electronic_file\raspi\Raspberry Pi 3294.ipt
- C:\Users\sbahn\Desktop\개인자료\Workspace\Python Workspace\고등학교 졸업과제\2학기\modeling\electronic_file\raspi\Raspberry Pi 3295.ipt
- C:\Users\sbahn\Desktop\개인자료\Workspace\Python Workspace\고등학교 졸업과제\2학기\modeling\electronic_file\raspi\Raspberry Pi 3296.ipt
- C:\Users\sbahn\Desktop\개인자료\Workspace\Python Workspace\고등학교 졸업과제\2학기\modeling\electronic_file\raspi\Raspberry Pi 3297.ipt
- C:\Users\sbahn\Desktop\개인자료\Workspace\Python Workspace\고등학교 졸업과제\2학기\modeling\electronic_file\raspi\Raspberry Pi 3298.ipt
- C:\Users\sbahn\Desktop\개인자료\Workspace\Python Workspace\고등학교 졸업과제\2학기\modeling\electronic_file\raspi\Raspberry Pi 3299.ipt
- C:\Users\sbahn\Desktop\개인자료\Workspace\Python Workspace\고등학교 졸업과제\2학기\modeling\electronic_file\raspi\Raspberry Pi 3300.ipt
- C:\Users\sbahn\Desktop\개인자료\Workspace\Python Workspace\고등학교 졸업과제\2학기\modeling\electronic_file\raspi\Raspberry Pi 3301.ipt
- C:\Users\sbahn\Desktop\개인자료\Workspace\Python Workspace\고등학교 졸업과제\2학기\modeling\electronic_file\raspi\Raspberry Pi 3302.ipt
- C:\Users\sbahn\Desktop\개인자료\Workspace\Python Workspace\고등학교 졸업과제\2학기\modeling\electronic_file\raspi\Raspberry Pi 3303.ipt
- C:\Users\sbahn\Desktop\개인자료\Workspace\Python Workspace\고등학교 졸업과제\2학기\modeling\electronic_file\raspi\Raspberry Pi 3304.ipt
- C:\Users\sbahn\Desktop\개인자료\Workspace\Python Workspace\고등학교 졸업과제\2학기\modeling\electronic_file\raspi\Raspberry Pi 3305.ipt
- C:\Users\sbahn\Desktop\개인자료\Workspace\Python Workspace\고등학교 졸업과제\2학기\modeling\electronic_file\raspi\Raspberry Pi 3306.ipt
- C:\Users\sbahn\Desktop\개인자료\Workspace\Python Workspace\고등학교 졸업과제\2학기\modeling\electronic_file\raspi\Raspberry Pi 3307.ipt
- C:\Users\sbahn\Desktop\개인자료\Workspace\Python Workspace\고등학교 졸업과제\2학기\modeling\electronic_file\raspi\Raspberry Pi 3308.ipt
- C:\Users\sbahn\Desktop\개인자료\Workspace\Python Workspace\고등학교 졸업과제\2학기\modeling\electronic_file\raspi\Raspberry Pi 3309.ipt
- C:\Users\sbahn\Desktop\개인자료\Workspace\Python Workspace\고등학교 졸업과제\2학기\modeling\electronic_file\raspi\Raspberry Pi 3310.ipt
- C:\Users\sbahn\Desktop\개인자료\Workspace\Python Workspace\고등학교 졸업과제\2학기\modeling\electronic_file\raspi\Raspberry Pi 3311.ipt
- C:\Users\sbahn\Desktop\개인자료\Workspace\Python Workspace\고등학교 졸업과제\2학기\modeling\electronic_file\raspi\Raspberry Pi 3312.ipt
- C:\Users\sbahn\Desktop\개인자료\Workspace\Python Workspace\고등학교 졸업과제\2학기\modeling\electronic_file\raspi\Raspberry Pi 3313.ipt
- C:\Users\sbahn\Desktop\개인자료\Workspace\Python Workspace\고등학교 졸업과제\2학기\modeling\electronic_file\raspi\Raspberry Pi 3314.ipt
- C:\Users\sbahn\Desktop\개인자료\Workspace\Python Workspace\고등학교 졸업과제\2학기\modeling\electronic_file\raspi\Raspberry Pi 3315.ipt
- C:\Users\sbahn\Desktop\개인자료\Workspace\Python Workspace\고등학교 졸업과제\2학기\modeling\electronic_file\raspi\Raspberry Pi 3316.ipt
- C:\Users\sbahn\Desktop\개인자료\Workspace\Python Workspace\고등학교 졸업과제\2학기\modeling\electronic_file\raspi\Raspberry Pi 3317.ipt
- C:\Users\sbahn\Desktop\개인자료\Workspace\Python Workspace\고등학교 졸업과제\2학기\modeling\electronic_file\raspi\Raspberry Pi 3318.ipt
- C:\Users\sbahn\Desktop\개인자료\Workspace\Python Workspace\고등학교 졸업과제\2학기\modeling\electronic_file\raspi\Raspberry Pi 3319.ipt
- C:\Users\sbahn\Desktop\개인자료\Workspace\Python Workspace\고등학교 졸업과제\2학기\modeling\electronic_file\raspi\Raspberry Pi 3320.ipt
- C:\Users\sbahn\Desktop\개인자료\Workspace\Python Workspace\고등학교 졸업과제\2학기\modeling\electronic_file\raspi\Raspberry Pi 3321.ipt
- C:\Users\sbahn\Desktop\개인자료\Workspace\Python Workspace\고등학교 졸업과제\2학기\modeling\electronic_file\raspi\Raspberry Pi 3322.ipt
- C:\Users\sbahn\Desktop\개인자료\Workspace\Python Workspace\고등학교 졸업과제\2학기\modeling\electronic_file\raspi\Raspberry Pi 3323.ipt
- C:\Users\sbahn\Desktop\개인자료\Workspace\Python Workspace\고등학교 졸업과제\2학기\modeling\electronic_file\raspi\Raspberry Pi 3324.ipt
- C:\Users\sbahn\Desktop\개인자료\Workspace\Python Workspace\고등학교 졸업과제\2학기\modeling\electronic_file\raspi\Raspberry Pi 3325.ipt
- C:\Users\sbahn\Desktop\개인자료\Workspace\Python Workspace\고등학교 졸업과제\2학기\modeling\electronic_file\raspi\Raspberry Pi 3326.ipt
- C:\Users\sbahn\Desktop\개인자료\Workspace\Python Workspace\고등학교 졸업과제\2학기\modeling\electronic_file\raspi\Raspberry Pi 3327.ipt
- C:\Users\sbahn\Desktop\개인자료\Workspace\Python Workspace\고등학교 졸업과제\2학기\modeling\electronic_file\raspi\Raspberry Pi 3328.ipt
- C:\Users\sbahn\Desktop\개인자료\Workspace\Python Workspace\고등학교 졸업과제\2학기\modeling\electronic_file\raspi\Raspberry Pi 3329.ipt
- C:\Users\sbahn\Desktop\개인자료\Workspace\Python Workspace\고등학교 졸업과제\2학기\modeling\electronic_file\raspi\Raspberry Pi 3330.ipt
- C:\Users\sbahn\Desktop\개인자료\Workspace\Python Workspace\고등학교 졸업과제\2학기\modeling\electronic_file\raspi\Raspberry Pi 3331.ipt
- C:\Users\sbahn\Desktop\개인자료\Workspace\Python Workspace\고등학교 졸업과제\2학기\modeling\electronic_file\raspi\Raspberry Pi 3332.ipt
- C:\Users\sbahn\Desktop\개인자료\Workspace\Python Workspace\고등학교 졸업과제\2학기\modeling\electronic_file\raspi\Raspberry Pi 3333.ipt
- C:\Users\sbahn\Desktop\개인자료\Workspace\Python Workspace\고등학교 졸업과제\2학기\modeling\electronic_file\raspi\Raspberry Pi 3334.ipt
- C:\Users\sbahn\Desktop\개인자료\Workspace\Python Workspace\고등학교 졸업과제\2학기\modeling\electronic_file\raspi\Raspberry Pi 3335.ipt
- C:\Users\sbahn\Desktop\개인자료\Workspace\Python Workspace\고등학교 졸업과제\2학기\modeling\electronic_file\raspi\Raspberry Pi 3336.ipt
- C:\Users\sbahn\Desktop\개인자료\Workspace\Python Workspace\고등학교 졸업과제\2학기\modeling\electronic_file\raspi\Raspberry Pi 3337.ipt
- C:\Users\sbahn\Desktop\개인자료\Workspace\Python Workspace\고등학교 졸업과제\2학기\modeling\electronic_file\raspi\Raspberry Pi 3338.ipt
- C:\Users\sbahn\Desktop\개인자료\Workspace\Python Workspace\고등학교 졸업과제\2학기\modeling\electronic_file\raspi\Raspberry Pi 3339.ipt
- C:\Users\sbahn\Desktop\개인자료\Workspace\Python Workspace\고등학교 졸업과제\2학기\modeling\electronic_file\raspi\Raspberry Pi 3340.ipt
- C:\Users\sbahn\Desktop\개인자료\Workspace\Python Workspace\고등학교 졸업과제\2학기\modeling\electronic_file\raspi\Raspberry Pi 3341.ipt
- C:\Users\sbahn\Desktop\개인자료\Workspace\Python Workspace\고등학교 졸업과제\2학기\modeling\electronic_file\raspi\Raspberry Pi 3342.ipt
- C:\Users\sbahn\Desktop\개인자료\Workspace\Python Workspace\고등학교 졸업과제\2학기\modeling\electronic_file\raspi\Raspberry Pi 3343.ipt
- C:\Users\sbahn\Desktop\개인자료\Workspace\Python Workspace\고등학교 졸업과제\2학기\modeling\electronic_file\raspi\Raspberry Pi 3344.ipt
- C:\Users\sbahn\Desktop\개인자료\Workspace\Python Workspace\고등학교 졸업과제\2학기\modeling\electronic_file\raspi\Raspberry Pi 3345.ipt
- C:\Users\sbahn\Desktop\개인자료\Workspace\Python Workspace\고등학교 졸업과제\2학기\modeling\electronic_file\raspi\Raspberry Pi 3346.ipt
- C:\Users\sbahn\Desktop\개인자료\Workspace\Python Workspace\고등학교 졸업과제\2학기\modeling\electronic_file\raspi\Raspberry Pi 3347.ipt
- C:\Users\sbahn\Desktop\개인자료\Workspace\Python Workspace\고등학교 졸업과제\2학기\modeling\electronic_file\raspi\Raspberry Pi 3348.ipt
- C:\Users\sbahn\Desktop\개인자료\Workspace\Python Workspace\고등학교 졸업과제\2학기\modeling\electronic_file\raspi\Raspberry Pi 3349.ipt
- C:\Users\sbahn\Desktop\개인자료\Workspace\Python Workspace\고등학교 졸업과제\2학기\modeling\electronic_file\raspi\Raspberry Pi 3350.ipt
- C:\Users\sbahn\Desktop\개인자료\Workspace\Python Workspace\고등학교 졸업과제\2학기\modeling\electronic_file\raspi\Raspberry Pi 3351.ipt
- C:\Users\sbahn\Desktop\개인자료\Workspace\Python Workspace\고등학교 졸업과제\2학기\modeling\electronic_file\raspi\Raspberry Pi 3352.ipt
- C:\Users\sbahn\Desktop\개인자료\Workspace\Python Workspace\고등학교 졸업과제\2학기\modeling\electronic_file\raspi\Raspberry Pi 3353.ipt
- C:\Users\sbahn\Desktop\개인자료\Workspace\Python Workspace\고등학교 졸업과제\2학기\modeling\electronic_file\raspi\Raspberry Pi 3354.ipt
- C:\Users\sbahn\Desktop\개인자료\Workspace\Python Workspace\고등학교 졸업과제\2학기\modeling\electronic_file\raspi\Raspberry Pi 3357.ipt
- C:\Users\sbahn\Desktop\개인자료\Workspace\Python Workspace\고등학교 졸업과제\2학기\modeling\electronic_file\raspi\Raspberry Pi 3355.ipt
- C:\Users\sbahn\Desktop\개인자료\Workspace\Python Workspace\고등학교 졸업과제\2학기\modeling\electronic_file\raspi\Raspberry Pi 3356.ipt
- C:\Users\sbahn\Desktop\개인자료\Workspace\Python Workspace\고등학교 졸업과제\2학기\modeling\electronic_file\raspi\Part2^Raspberry Pi 3.ipt
- C:\Users\sbahn\Desktop\개인자료\Workspace\Python Workspace\고등학교 졸업과제\2학기\modeling\electronic_file\raspi\Raspberry Pi 3360.ipt
- C:\Users\sbahn\Desktop\개인자료\Workspace\Python Workspace\고등학교 졸업과제\2학기\modeling\electronic_file\raspi\Part4^Raspberry Pi 3.ipt
- C:\Users\sbahn\Desktop\개인자료\Workspace\Python Workspace\고등학교 졸업과제\2학기\modeling\electronic_file\raspi\Solder2.ipt
- C:\Users\sbahn\Desktop\개인자료\Workspace\Python Workspace\고등학교 졸업과제\2학기\modeling\electronic_file\raspi\Raspberry Pi 3358.ipt
- C:\Users\sbahn\Desktop\개인자료\Workspace\Python Workspace\고등학교 졸업과제\2학기\modeling\electronic_file\raspi\Raspberry Pi 3359.ipt
- C:\Users\sbahn\Desktop\개인자료\Workspace\Python Workspace\고등학교 졸업과제\2학기\modeling\electronic_file\raspi\mf-msmf050-2.ipt
- C:\Users\sbahn\Desktop\개인자료\Workspace\Python Workspace\고등학교 졸업과제\2학기\modeling\electronic_file\raspi\Raspberry Pi 3163_smaller.ipt
- C:\Users\sbahn\Desktop\개인자료\Workspace\Python Workspace\고등학교 졸업과제\2학기\modeling\electronic_file\raspi\Raspberry Pi 353_smaller.ipt
- C:\Users\sbahn\Desktop\개인자료\Workspace\Python Workspace\고등학교 졸업과제\2학기\modeling\electronic_file\raspi\Raspberry Pi 3164_small.ipt
- C:\Users\sbahn\Desktop\개인자료\Workspace\Python Workspace\고등학교 졸업과제\2학기\modeling\electronic_file\raspi\Raspberry Pi 3165_smaller.ipt
- C:\Users\sbahn\Desktop\개인자료\Workspace\Python Workspace\고등학교 졸업과제\2학기\modeling\electronic_file\raspi\Raspberry Pi 3141_smaller.ipt
- C:\Users\sbahn\Desktop\개인자료\Workspace\Python Workspace\고등학교 졸업과제\2학기\modeling\electronic_file\raspi\Assem1^Raspberry Pi 3.iam
- C:\Users\sbahn\Desktop\개인자료\Workspace\Python Workspace\고등학교 졸업과제\2학기\modeling\electronic_file\raspi\raspberry_pi_B+_(microsd2).ipt
## Components (634 placed, 323 different names)
1. Raspberry Pi 3157:1
2. Raspberry Pi 3242:1
3. Raspberry Pi 3266:1
4. raspberry_pi_3(bar_180_2x20):2
5. RPi3_ModelB v1:1 [sub-assembly]
6. Raspberry Pi 312:1
7. Raspberry Pi 314:1
8. Raspberry Pi 3172:1
9. Raspberry Pi 3173:1
10. Raspberry Pi 3174:1
11. Raspberry Pi 3175:1
12. Raspberry Pi 3176:1
13. Raspberry Pi 3177:1
14. Raspberry Pi 3178:1
15. Raspberry Pi 3179:1
16. Raspberry Pi 3180:1
17. Raspberry Pi 3181:1
18. Raspberry Pi 3182:1
19. Raspberry Pi 3183:1
20. Raspberry Pi 3184:1
21. Raspberry Pi 3185:1
22. Raspberry Pi 3186:1
23. Raspberry Pi 3187:1
24. Raspberry Pi 3188:1
25. Raspberry Pi 3189:1
26. Raspberry Pi 3190:1
27. Raspberry Pi 3191:1
28. Raspberry Pi 3192:1
29. Raspberry Pi 3193:1
30. Raspberry Pi 3194:1
31. Raspberry Pi 3195:1
32. Raspberry Pi 3196:1
33. Raspberry Pi 3197:1
34. Raspberry Pi 3198:1
35. Raspberry Pi 3199:1
36. Raspberry Pi 3200:1
37. Raspberry Pi 3201:1
38. Raspberry Pi 3202:1
39. Raspberry Pi 3203:1
40. Raspberry Pi 3204:1
41. Raspberry Pi 3205:1
42. Raspberry Pi 3206:1
43. Raspberry Pi 3207:1
44. Raspberry Pi 3208:1
45. Raspberry Pi 3209:1
46. Raspberry Pi 3210:1
47. Raspberry Pi 3211:1
48. Raspberry Pi 3212:1
49. Raspberry Pi 3213:1
50. Raspberry Pi 3214:1
51. Raspberry Pi 3215:1
52. Raspberry Pi 3216:1
53. Raspberry Pi 3217:1
54. Raspberry Pi 3218:1
55. Raspberry Pi 3219:1
56. Raspberry Pi 3220:1
57. Raspberry Pi 3221:1
58. Raspberry Pi 3222:1
59. Raspberry Pi 3223:1
60. Raspberry Pi 3224:1
61. Raspberry Pi 3225:1
62. Raspberry Pi 3226:1
63. Raspberry Pi 3227:1
64. Raspberry Pi 3228:1
65. Raspberry Pi 3229:1
66. Raspberry Pi 3230:1
67. Raspberry Pi 3231:1
68. Raspberry Pi 3232:1
69. Raspberry Pi 3233:1
70. Raspberry Pi 3234:1
71. Raspberry Pi 3235:1
72. Raspberry Pi 31:1
73. Raspberry Pi 36:1
74. Raspberry Pi 32:1
75. Raspberry Pi 33:1
76. Raspberry Pi 34:1
77. Raspberry Pi 35:1
78. Raspberry Pi 37:1
79. Raspberry Pi 38:1
80. Raspberry Pi 39:1
81. Raspberry Pi 310:1
82. Raspberry Pi 311:1
83. Raspberry Pi 313:1
84. Raspberry Pi 315:1
85. Raspberry Pi 316:1
86. Raspberry Pi 317:1
87. Raspberry Pi 318:1
88. Raspberry Pi 319:1
89. Raspberry Pi 320:1
90. Raspberry Pi 322:1
91. Raspberry Pi 323:1
92. Raspberry Pi 324:1
93. Raspberry Pi 325:1
94. Raspberry Pi 326:1
95. Raspberry Pi 327:1
96. Raspberry Pi 328:1
97. Raspberry Pi 329:1
98. Raspberry Pi 330:1
99. Raspberry Pi 331:1
100. Raspberry Pi 332:1
101. Raspberry Pi 333:1
102. Raspberry Pi 334:1
103. Raspberry Pi 335:1
104. Raspberry Pi 336:1
105. Raspberry Pi 337:1
106. Raspberry Pi 338:1
107. Raspberry Pi 339:1
108. Raspberry Pi 340:1
109. Raspberry Pi 341:1
110. Raspberry Pi 342:1
111. Raspberry Pi 343:1
112. Raspberry Pi 344:1
113. Raspberry Pi 345:1
114. Raspberry Pi 346:1
115. Raspberry Pi 347:1
116. Raspberry Pi 348:1
117. Raspberry Pi 349:1
118. Raspberry Pi 350:1
119. Raspberry Pi 351:1
120. Raspberry Pi 352:1
121. Raspberry Pi 353:1
122. Raspberry Pi 354:1
123. Raspberry Pi 355:1
124. Raspberry Pi 356:1
125. Raspberry Pi 357:1
126. Raspberry Pi 358:1
127. Raspberry Pi 359:1
128. Raspberry Pi 360:1
129. Raspberry Pi 361:1
130. Raspberry Pi 362:1
131. Raspberry Pi 363:1
132. Raspberry Pi 364:1
133. Raspberry Pi 365:1
134. Raspberry Pi 366:1
135. Raspberry Pi 367:1
136. Raspberry Pi 368:1
137. Raspberry Pi 369:1
138. Raspberry Pi 370:1
139. Raspberry Pi 371:1
140. Raspberry Pi 372:1
141. Raspberry Pi 373:1
142. Raspberry Pi 374:1
143. Raspberry Pi 375:1
144. Raspberry Pi 376:1
145. Raspberry Pi 377:1
146. Raspberry Pi 378:1
147. Raspberry Pi 379:1
148. Raspberry Pi 380:1
149. Raspberry Pi 381:1
150. Raspberry Pi 382:1
151. Raspberry Pi 383:1
152. Raspberry Pi 385:1
153. Raspberry Pi 386:1
154. Raspberry Pi 387:1
155. Raspberry Pi 388:1
156. Raspberry Pi 390:1
157. Raspberry Pi 391:1
158. Raspberry Pi 393:1
159. Raspberry Pi 394:1
160. Raspberry Pi 395:1
161. Raspberry Pi 396:1
162. Raspberry Pi 397:1
163. Raspberry Pi 398:1
164. Raspberry Pi 399:1
165. Raspberry Pi 3100:1
166. Raspberry Pi 3101:1
167. Raspberry Pi 3102:1
168. Raspberry Pi 3103:1
169. Raspberry Pi 3104:1
170. Raspberry Pi 3105:1
171. Raspberry Pi 3106:1
172. Raspberry Pi 3107:1
173. Raspberry Pi 3108:1
174. Raspberry Pi 3109:1
175. Raspberry Pi 3110:1
176. Raspberry Pi 3111:1
177. Raspberry Pi 3112:1
178. Raspberry Pi 3113:1
179. Raspberry Pi 3114:1
180. Raspberry Pi 3115:1
181. Raspberry Pi 3116:1
182. Raspberry Pi 3117:1
183. Raspberry Pi 3118:1
184. Raspberry Pi 3119:1
185. Raspberry Pi 3120:1
186. Raspberry Pi 3121:1
187. Raspberry Pi 3122:1
188. Raspberry Pi 3123:1
189. Raspberry Pi 3124:1
190. Raspberry Pi 3125:1
191. Raspberry Pi 3126:1
192. Raspberry Pi 3127:1
193. Raspberry Pi 3128:1
194. Raspberry Pi 3129:1
195. Raspberry Pi 3130:1
196. Raspberry Pi 3131:1
197. Raspberry Pi 3132:1
198. Raspberry Pi 3133:1
199. Raspberry Pi 3134:1
200. Raspberry Pi 3135:1
201. Raspberry Pi 3137:1
202. Raspberry Pi 3138:1
203. Raspberry Pi 3139:1
204. Raspberry Pi 3140:1
205. Raspberry Pi 3141:1
206. Raspberry Pi 3142:1
207. Raspberry Pi 3143:1
208. Raspberry Pi 3144:1
209. Raspberry Pi 3146:1
210. Raspberry Pi 3147:1
211. Raspberry Pi 3149:1
212. Raspberry Pi 3150:1
213. Raspberry Pi 3151:1
214. Raspberry Pi 3152:1
215. Raspberry Pi 3153:1
216. Raspberry Pi 3154:1
217. Raspberry Pi 3155:1
218. Raspberry Pi 3156:1
219. Raspberry Pi 3158:1
220. Raspberry Pi 3159:1
221. Raspberry Pi 3160:1
222. Raspberry Pi 3161:1
223. Raspberry Pi 3162:1
224. Raspberry Pi 3163:1
225. Raspberry Pi 3164:1
226. Raspberry Pi 3165:1
227. Raspberry Pi 3166:1
228. Raspberry Pi 3167:1
229. Raspberry Pi 3168:1
230. Raspberry Pi 3169:1
231. Raspberry Pi 3170:1
232. Raspberry Pi 3171:1
233. Raspberry Pi 3276:1
234. Raspberry Pi 3277:1
235. Raspberry Pi 3278:1
236. Raspberry Pi 3279:1
237. Raspberry Pi 3280:1
238. Raspberry Pi 3281:1
239. Raspberry Pi 3282:1
240. Raspberry Pi 3283:1
241. Raspberry Pi 3284:1
242. Raspberry Pi 3285:1
243. Raspberry Pi 3286:1
244. Raspberry Pi 3287:1
245. Raspberry Pi 3288:1
246. Raspberry Pi 3289:1
247. Raspberry Pi 3290:1
248. Raspberry Pi 3291:1
249. Raspberry Pi 3292:1
250. Raspberry Pi 3293:1
251. Raspberry Pi 3294:1
252. Raspberry Pi 3295:1
253. Raspberry Pi 3296:1
254. Raspberry Pi 3297:1
255. Raspberry Pi 3298:1
256. Raspberry Pi 3299:1
257. Raspberry Pi 3300:1
258. Raspberry Pi 3301:1
259. Raspberry Pi 3302:1
260. Raspberry Pi 3303:1
261. Raspberry Pi 3304:1
262. Raspberry Pi 3305:1
263. Raspberry Pi 3306:1
264. Raspberry Pi 3307:1
265. Raspberry Pi 3308:1
266. Raspberry Pi 3309:1
267. Raspberry Pi 3310:1
268. Raspberry Pi 3311:1
269. Raspberry Pi 3312:1
270. Raspberry Pi 3313:1
271. Raspberry Pi 3314:1
272. Raspberry Pi 3315:1
273. Raspberry Pi 3316:1
274. Raspberry Pi 3317:1
275. Raspberry Pi 3318:1
276. Raspberry Pi 3319:1
277. Raspberry Pi 3320:1
278. Raspberry Pi 3321:1
279. Raspberry Pi 3322:1
280. Raspberry Pi 3323:1
281. Raspberry Pi 3324:1
282. Raspberry Pi 3325:1
283. Raspberry Pi 3326:1
284. Raspberry Pi 3327:1
285. Raspberry Pi 3328:1
286. Raspberry Pi 3329:1
287. Raspberry Pi 3330:1
288. Raspberry Pi 3331:1
289. Raspberry Pi 3332:1
290. Raspberry Pi 3333:1
291. Raspberry Pi 3334:1
292. Raspberry Pi 3335:1
293. Raspberry Pi 3336:1
294. Raspberry Pi 3337:1
295. Raspberry Pi 3338:1
296. Raspberry Pi 3339:1
297. Raspberry Pi 3340:1
298. Raspberry Pi 3341:1
299. Raspberry Pi 3342:1
300. Raspberry Pi 3343:1
301. Raspberry Pi 3344:1
302. Raspberry Pi 3345:1
303. Raspberry Pi 3346:1
304. Raspberry Pi 3347:1
305. Raspberry Pi 3348:1
306. Raspberry Pi 3349:1
307. Raspberry Pi 3350:1
308. Raspberry Pi 3351:1
309. Raspberry Pi 3352:1
310. Raspberry Pi 3353:1
311. Raspberry Pi 3354:1
312. Raspberry Pi 327:2
313. Raspberry Pi 340:2
314. Raspberry Pi 344:2
315. Raspberry Pi 344:3
316. Raspberry Pi 340:3
317. Raspberry Pi 344:4
318. Raspberry Pi 340:4
319. Raspberry Pi 344:6
320. Raspberry Pi 340:6
321. Raspberry Pi 344:7
322. Raspberry Pi 340:7
323. Raspberry Pi 340:8
324. Raspberry Pi 344:8
325. Raspberry Pi 340:9
326. Raspberry Pi 344:9
327. Raspberry Pi 3357:1
328. Raspberry Pi 3355:1
329. Raspberry Pi 3356:1
330. Raspberry Pi 374:2
331. Raspberry Pi 3141:2
332. Raspberry Pi 374:3
333. Raspberry Pi 374:4
334. Raspberry Pi 374:5
335. Part2^Raspberry Pi 3:1
336. Raspberry Pi 3360:1
337. Part4^Raspberry Pi 3:1
338. Raspberry Pi 3159:2
339. Raspberry Pi 3158:2
340. Raspberry Pi 3160:2
341. Raspberry Pi 3162:2
342. Raspberry Pi 3161:2
343. Raspberry Pi 359:2
344. Raspberry Pi 3165:2
345. Raspberry Pi 353:2
346. Raspberry Pi 3164:2
347. Raspberry Pi 3163:2
348. Raspberry Pi 355:3
349. Raspberry Pi 3168:3
350. Raspberry Pi 3170:3
351. Raspberry Pi 3169:3
352. Raspberry Pi 3171:3
353. Raspberry Pi 3167:3
354. Raspberry Pi 3166:3
355. Raspberry Pi 353:3
356. Raspberry Pi 3165:3